# Autodesk Inventor assembly: OpenRaman.V1
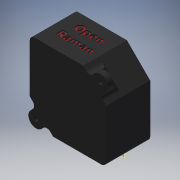
[picture p0: Inventor's stored thumbnail of the model, 180x180]
Saved by Autodesk Inventor 2017 (Build 210142000, 142)
## iProperties
Created: 2017-08-01
Part Number: OpenRaman.V1
Document SubType Name: Assembly
Designer: vmiguel
Author: vmiguel
## Documents named in this file (6)
- C:\Users\vmiguel\Dropbox\OpenRaman\OpenRaman\Hardware\OpenRaman.V1.iam
- C:\Users\vmiguel\Dropbox\OpenRaman\OpenRaman\Hardware\3D Printed Parts\CorpoPrismatico.ipt
- C:\Users\vmiguel\Dropbox\OpenRaman\OpenRaman\Hardware\Supriments\TCD1304AP.ipt
- C:\Users\vmiguel\Dropbox\OpenRaman\OpenRaman\Hardware\Supriments\Prisma-25.4.ipt
- C:\Users\vmiguel\Dropbox\OpenRaman\OpenRaman\Hardware\Supriments\Prisma-90.ipt
- C:\Users\vmiguel\Dropbox\OpenRaman\OpenRaman\Hardware\Supriments\Prisma-12.7.ipt
## Components (5 placed, 5 different names)
1. CorpoPrismatico:1 — Mate:2, Mate:3, Mate:4, Mate:5, Mate:6, Mate:7, Mate:8, Mate:9, Mate:10, Mate:11, Flush:1
2. TCD1304AP:1 — Mate:11, Flush:1
3. Prisma-25.4:1 — Mate:2, Mate:3, Mate:4
4. Prisma-90:1 — Mate:5, Mate:6, Mate:7
5. Prisma-12.7:1 — Mate:8, Mate:9, Mate:10
## Relationships (11: Mate 10, Flush 1)
- Mate:2: CorpoPrismatico:1 ↔ Prisma-25.4:1
- Mate:3: CorpoPrismatico:1 ↔ Prisma-25.4:1
- Mate:4: CorpoPrismatico:1 ↔ Prisma-25.4:1
- Mate:5: CorpoPrismatico:1 ↔ Prisma-90:1
- Mate:6: CorpoPrismatico:1 ↔ Prisma-90:1
- Mate:7: CorpoPrismatico:1 ↔ Prisma-90:1
- Mate:8: CorpoPrismatico:1 ↔ Prisma-12.7:1
- Mate:9: CorpoPrismatico:1 ↔ Prisma-12.7:1
- Mate:10: CorpoPrismatico:1 ↔ Prisma-12.7:1
- Mate:11 (0.5 mm): CorpoPrismatico:1 ↔ TCD1304AP:1
- Flush:1: CorpoPrismatico:1 ↔ TCD1304AP:1
